# Autodesk Inventor assembly: back_box_asembly
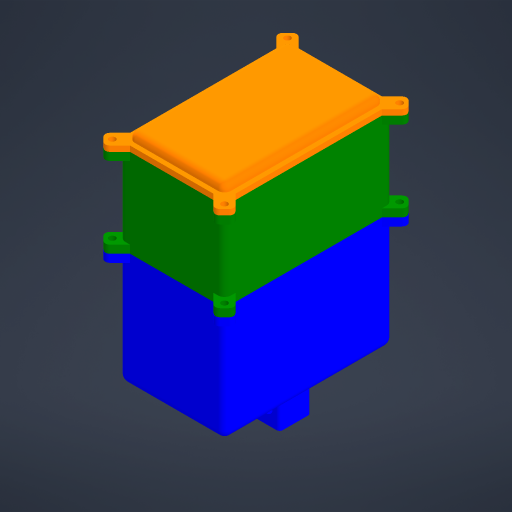
[picture p0: Inventor's stored thumbnail of the model, 512x512]
Saved by Autodesk Inventor 2024 (Build 280153000, 153)
## iProperties
Created: 2023-05-15
Part Number: back_box_asembly
Document SubType Name: Assembly
Designer: user
Author: user
## Documents named in this file (6)
- D:\Docs\Robot\3d\machine_body\back_box_asembly.iam
- D:\Docs\Robot\3d\machine_body\back_box_asembly\back_box.ipt
- D:\Docs\Robot\3d\electronics\Battery_18650_asembly.iam
- D:\Docs\Robot\3d\electronics\BTS7960\BTS7960.iam
- D:\Docs\Robot\3d\machine_body\back_box_asembly\back_box_mid.ipt
- D:\Docs\Robot\3d\machine_body\back_box_asembly\back_box_cup.ipt
## Components (6 placed, 5 different names)
1. back_box:1 — Совмещение:1, Совмещение:2, Совмещение:3, Совмещение:4, Совмещение:5, Касательность:1, Касательность:2, Касательность:3, Касательность:4, Заподлицо:1
2. Battery_18650_asembly:1 [sub-assembly] — Совмещение:5, Касательность:1, Касательность:2, Касательность:3, Касательность:4
3. BTS7960:1 [sub-assembly] — Совмещение:6, Заподлицо:2, Заподлицо:3, Совмещение:8, Совмещение:9
4. back_box_mid:1 — Заподлицо:1, Совмещение:6, Совмещение:7, Совмещение:8, Совмещение:9, Заподлицо:4
5. BTS7960:2 [sub-assembly] — Совмещение:7, Заподлицо:2, Заподлицо:3
6. back_box_cup:1 — Заподлицо:4
## Relationships (17: Mate 9, Tangent 4, Flush 4)
- Совмещение:1 [Mate]: back_box:1
- Совмещение:2 [Mate]: back_box:1
- Совмещение:3 [Mate]: back_box:1
- Совмещение:4 [Mate]: back_box:1
- Совмещение:5 [Mate]: back_box:1 ↔ Battery_18650_asembly:1
- Касательность:1 [Tangent] (5 mm): back_box:1 ↔ Battery_18650_asembly:1
- Касательность:2 [Tangent] (5 mm): back_box:1 ↔ Battery_18650_asembly:1
- Касательность:3 [Tangent] (5 mm): back_box:1 ↔ Battery_18650_asembly:1
- Касательность:4 [Tangent] (5 mm): back_box:1 ↔ Battery_18650_asembly:1
- Заподлицо:1 [Flush]: back_box:1 ↔ back_box_mid:1
- Совмещение:6 [Mate]: BTS7960:1 ↔ back_box_mid:1
- Совмещение:7 [Mate]: back_box_mid:1 ↔ BTS7960:2
- Заподлицо:2 [Flush]: BTS7960:1 ↔ BTS7960:2
- Заподлицо:3 [Flush]: BTS7960:1 ↔ BTS7960:2
- Совмещение:8 [Mate] (8 mm): BTS7960:1 ↔ back_box_mid:1
- Совмещение:9 [Mate] (1 mm): BTS7960:1 ↔ back_box_mid:1
- Заподлицо:4 [Flush]: back_box_mid:1 ↔ back_box_cup:1
